# Autodesk Inventor assembly: Wedge
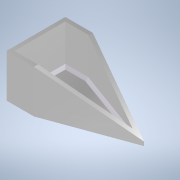
[picture p0: Inventor's stored thumbnail of the model, 180x180]
Saved by Autodesk Inventor 2020 (Build 240168000, 168)
## iProperties
Created: 2020-01-30
Part Number: Wedge
Document SubType Name: Weldment
Designer: Connor
Weld Material: Aluminum 6061, Welded
Author: Connor
## Documents named in this file (3)
- C:\Users\Connor\Desktop\KSU\RMC\Wedge.iam
- C:\Users\Connor\Desktop\KSU\RMC\Wedge_base.ipt
- C:\Users\Connor\Desktop\KSU\RMC\Wedge_wall.ipt
## Components (2 placed, 2 different names)
1. Wedge_base:1 — Mate:1, Mate:2
2. Wedge_wall:1 — Mate:1, Mate:2
## Relationships (2: Mate 2)
- Mate:1: Wedge_base:1 ↔ Wedge_wall:1
- Mate:2: Wedge_base:1 ↔ Wedge_wall:1
